# Autodesk Inventor assembly: LightRail_assembly
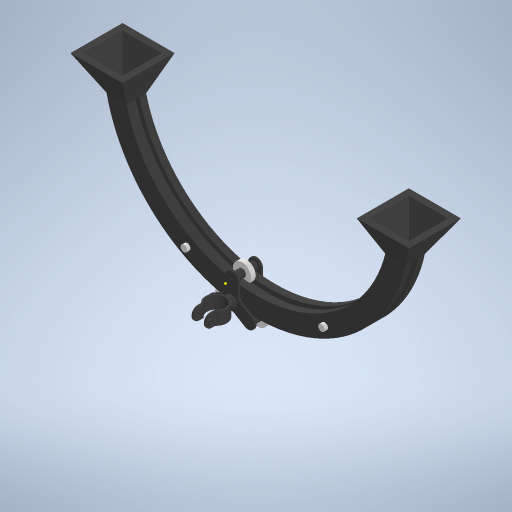
[picture p0: Inventor's stored thumbnail of the model, 512x512]
Saved by Autodesk Inventor 2023 (Build 270158000, 158)
## iProperties
Created: 2023-04-29
Part Number: LightRail_assembly
Document SubType Name: Assembly
Designer: ringl
Author: ringl
## Documents named in this file (6)
- C:\Users\ringl\Documents\Uni Classes\Y3S2\EE318-Project\EE318-Project\CAD\LightRail\LightRail_assembly.iam
- C:\Users\ringl\Documents\Uni Classes\Y3S2\EE318-Project\EE318-Project\CAD\LightRail\LightRail_endSection.ipt
- C:\Users\ringl\Documents\Uni Classes\Y3S2\EE318-Project\EE318-Project\CAD\LightRail\LightRail_middleSection.ipt
- C:\Users\ringl\Documents\Uni Classes\Y3S2\EE318-Project\EE318-Project\CAD\LightRail\LightRail_intermediateSection.ipt
- C:\Users\ringl\Documents\Uni Classes\Y3S2\EE318-Project\EE318-Project\CAD\LightRail\Pin.ipt
- C:\Users\ringl\Documents\Uni Classes\Y3S2\EE318-Project\EE318-Project\CAD\LightCart\LigthtCart-assembly.iam
## Components (8 placed, 5 different names)
1. LightRail_endSection:1 — Flush:1, Mate:1, Mate:2
2. LightRail_intermediateSection:1 — Flush:1, Mate:1, Mate:2, Flush:2, Mate:3, Mate:4
3. LightRail_middleSection:1 — Flush:2, Mate:3, Mate:4, Flush:3, Mate:5, Mate:6, Mate:10, Mate:11, Mate:12, Mate:13
4. LightRail_intermediateSection:2 — Flush:3, Mate:5, Mate:6, Flush:4, Mate:7, Mate:8, Mate:9
5. LightRail_endSection:2 — Flush:4, Mate:7, Mate:8
6. Pin:1 — Mate:9, Mate:10
7. Pin:2 — Mate:11, Mate:12
8. LigthtCart-assembly:1 [sub-assembly] — Mate:13
## Relationships (17: Mate 13, Flush 4)
- Flush:1: LightRail_endSection:1 ↔ LightRail_intermediateSection:1
- Mate:1: LightRail_endSection:1 ↔ LightRail_intermediateSection:1
- Mate:2: LightRail_endSection:1 ↔ LightRail_intermediateSection:1
- Flush:2: LightRail_intermediateSection:1 ↔ LightRail_middleSection:1
- Mate:3: LightRail_intermediateSection:1 ↔ LightRail_middleSection:1
- Mate:4: LightRail_intermediateSection:1 ↔ LightRail_middleSection:1
- Flush:3: LightRail_middleSection:1 ↔ LightRail_intermediateSection:2
- Mate:5: LightRail_middleSection:1 ↔ LightRail_intermediateSection:2
- Mate:6: LightRail_middleSection:1 ↔ LightRail_intermediateSection:2
- Flush:4: LightRail_intermediateSection:2 ↔ LightRail_endSection:2
- Mate:7: LightRail_intermediateSection:2 ↔ LightRail_endSection:2
- Mate:8: LightRail_intermediateSection:2 ↔ LightRail_endSection:2
- Mate:9: LightRail_intermediateSection:2 ↔ Pin:1
- Mate:10: LightRail_middleSection:1 ↔ Pin:1
- Mate:11: LightRail_middleSection:1 ↔ Pin:2
- Mate:12: LightRail_middleSection:1 ↔ Pin:2
- Mate:13 (1 mm): LightRail_middleSection:1 ↔ LigthtCart-assembly:1
